# Autodesk Inventor assembly: Eslabon1
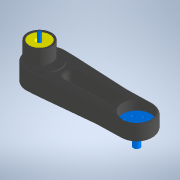
[picture p0: Inventor's stored thumbnail of the model, 180x180]
Saved by Autodesk Inventor 2021 (Build 250183000, 183)
## iProperties
Created: 2022-04-22
Part Number: Eslabon1
Document SubType Name: Assembly
Designer: Alcatraz
Author: Alcatraz
## Documents named in this file (7)
- F:\Tesis\TESIS\Matlab\Pruebas\Prueba3_Simulacion2\Eslabon1.iam
- F:\Tesis\TESIS\Eslabon_9_Parametrizado.ipt
- F:\Tesis\TESIS\Eje_3_parametrizado.ipt
- F:\Tesis\TESIS\AX-12A,18A,12W,MX-12W(stp)\AX-12A.iam
- F:\Tesis\TESIS\Tapa_eslabon.ipt
- F:\Tesis\TESIS\Brida_5_parametrizado.ipt
- F:\Tesis\TESIS\rodamiento_dummie.ipt
## Components (7 placed, 6 different names)
1. Eslabon_9_Parametrizado:1 — Coincidencia:1, Coincidencia:2, Coincidencia:3, Coincidencia:7, Coincidencia:8, Coincidencia:9, Coincidencia:12
2. Eje_3_parametrizado:1 — Coincidencia:1, Coincidencia:2, Coincidencia:3
3. AX-12A:1 [sub-assembly] — Coincidencia:4, Coincidencia:5, Coincidencia:6, Coincidencia:13, Coincidencia:14, Coincidencia:15
4. Tapa_eslabon:1 — Coincidencia:4, Coincidencia:5, Coincidencia:6, Coincidencia:7, Coincidencia:8, Coincidencia:9
5. Brida_5_parametrizado:1 — Coincidencia:13, Coincidencia:14, Coincidencia:15, Coincidencia:16
6. rodamiento_dummie:1 — Coincidencia:10, Coincidencia:11, Coincidencia:12
7. rodamiento_dummie:2 — Coincidencia:10, Coincidencia:11, Coincidencia:16
## Relationships (16: Mate 16)
- Coincidencia:1 [Mate]: Eslabon_9_Parametrizado:1 ↔ Eje_3_parametrizado:1
- Coincidencia:2 [Mate]: Eslabon_9_Parametrizado:1 ↔ Eje_3_parametrizado:1
- Coincidencia:3 [Mate]: Eslabon_9_Parametrizado:1 ↔ Eje_3_parametrizado:1
- Coincidencia:4 [Mate]: AX-12A:1 ↔ Tapa_eslabon:1
- Coincidencia:5 [Mate]: AX-12A:1 ↔ Tapa_eslabon:1
- Coincidencia:6 [Mate]: AX-12A:1 ↔ Tapa_eslabon:1
- Coincidencia:7 [Mate]: Eslabon_9_Parametrizado:1 ↔ Tapa_eslabon:1
- Coincidencia:8 [Mate]: Eslabon_9_Parametrizado:1 ↔ Tapa_eslabon:1
- Coincidencia:9 [Mate]: Eslabon_9_Parametrizado:1 ↔ Tapa_eslabon:1
- Coincidencia:10 [Mate]: rodamiento_dummie:1 ↔ rodamiento_dummie:2
- Coincidencia:11 [Mate]: rodamiento_dummie:1 ↔ rodamiento_dummie:2
- Coincidencia:12 [Mate]: Eslabon_9_Parametrizado:1 ↔ rodamiento_dummie:1
- Coincidencia:13 [Mate]: AX-12A:1 ↔ Brida_5_parametrizado:1
- Coincidencia:14 [Mate]: AX-12A:1 ↔ Brida_5_parametrizado:1
- Coincidencia:15 [Mate]: AX-12A:1 ↔ Brida_5_parametrizado:1
- Coincidencia:16 [Mate]: Brida_5_parametrizado:1 ↔ rodamiento_dummie:2
